# Autodesk Inventor assembly: Ensemble côté suspension
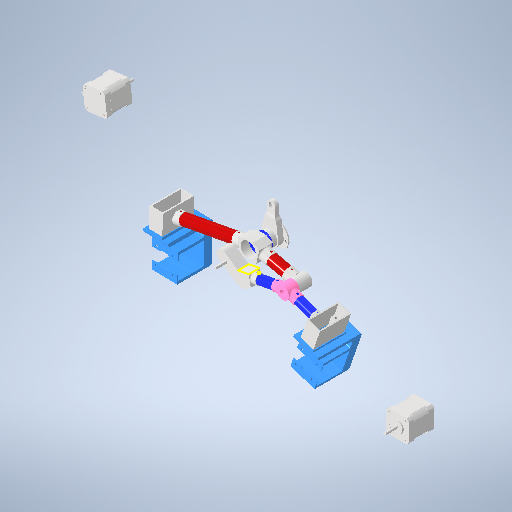
[picture p0: Inventor's stored thumbnail of the model, 512x512]
Saved by Autodesk Inventor 2026.2 (Build 302298010, 298A)
## iProperties
Created: 2026-03-16
Part Number: Ensemble côté suspension
Document SubType Name: Assembly
Designer: genon
Author: genon
## Documents named in this file (16)
- C:\Users\genon\Documents\Henallux Passerelle\Projet de conception\Cassini T-X\Inventor\Suspension\Ensemble côté suspension.iam
- C:\Users\genon\Documents\Henallux Passerelle\Projet de conception\Cassini T-X\Inventor\Suspension\bièlle côté.ipt
- C:\Users\genon\Documents\Henallux Passerelle\Projet de conception\Cassini T-X\Inventor\Suspension\bielle côté 2.ipt
- C:\Users\genon\Documents\Henallux Passerelle\Projet de conception\Cassini T-X\Inventor\Suspension\bielle côté 3.ipt
- C:\Users\genon\Documents\Henallux Passerelle\Projet de conception\Cassini T-X\Inventor\Suspension\bielle côté 0.ipt
- C:\Users\genon\Documents\Henallux Passerelle\Projet de conception\Cassini T-X\Inventor\Suspension\Rolling v2.ipt
- C:\Users\genon\Documents\Henallux Passerelle\Projet de conception\Cassini T-X\Inventor\Suspension\tubelong_rocker.ipt
- C:\Users\genon\Documents\Henallux Passerelle\Projet de conception\Cassini T-X\Inventor\Suspension\tube vers bogie.ipt
- C:\Users\genon\Documents\Henallux Passerelle\Projet de conception\Cassini T-X\Inventor\Suspension\bielle rocker.ipt
- C:\Users\genon\Documents\Henallux Passerelle\Projet de conception\Cassini T-X\Inventor\Suspension\bielle rocker2.ipt
- C:\Users\genon\Documents\Henallux Passerelle\Projet de conception\Cassini T-X\Inventor\Suspension\bielle roue milieu.ipt
- C:\Users\genon\Documents\Henallux Passerelle\Projet de conception\Cassini T-X\Inventor\Suspension\Attache moteur.ipt
- C:\Users\genon\Documents\Henallux Passerelle\Projet de conception\Cassini T-X\Inventor\Suspension\tube des bogies.ipt
- C:\Users\genon\Documents\Henallux Passerelle\Projet de conception\Cassini T-X\Inventor\Composants\NEMA17_17HS19-2004S1_Stepperonline.ipt
- C:\Users\genon\Documents\Henallux Passerelle\Projet de conception\Cassini T-X\Inventor\Suspension\Attache servomoteur.ipt
- C:\Users\genon\Documents\Henallux Passerelle\Projet de conception\Cassini T-X\Inventor\Suspension\Attache servomoteur_bogie.ipt
## Components (21 placed, 15 different names)
1. bièlle côté:1 — Placage:10, Placage:11, Placage:12, Placage:13, Placage:14, Placage:17, Placage:18, Placage:19
2. bielle côté 2:1 — Placage:8, Placage:9, Placage:15, Placage:16, Placage:17, Placage:18
3. bielle côté 3:1 — Placage:15, Placage:16, Cylindrique:1, Cylindrique:7, Placage:32, Placage:41
4. bielle côté 0:1 — Placage:12
5. Rolling v2:2 — Placage:8, Placage:9, Placage:19
6. Rolling v2:3 — Placage:10, Placage:11
7. bielle côté 0:2 — Placage:13, Placage:14
8. tubelong_rocker:1 — Cylindrique:1, Placage:41, Placage:42, Placage:43
9. tube vers bogie:1 — Cylindrique:7, Placage:32, Cylindrique:8, Placage:33
10. bielle rocker2:1 — Placage:31, Cylindrique:9, Placage:34, Cylindrique:10, Placage:35, Cylindrique:13
11. bielle roue milieu:1 — Cylindrique:11, Placage:36
12. bielle rocker:1 — Placage:29, Placage:31, Cylindrique:8, Placage:33, Cylindrique:12, Cylindrique:13
13. Rolling v2:4 — Placage:29, Cylindrique:12
14. tube des bogies:1 — Cylindrique:9, Placage:34, Cylindrique:11, Placage:36
15. tube des bogies:2 — Cylindrique:10, Placage:35, Placage:44, Placage:45
16. NEMA17_17HS19-2004S1_Stepperonline:1
17. NEMA17_17HS19-2004S1_Stepperonline:2
18. Attache servomoteur:1 — Placage:42, Placage:43, Placage:46, Placage:47, Placage:48
19. Attache servomoteur_bogie:1 — Placage:44, Placage:45, Placage:49, Placage:50, Placage:51
20. Attache moteur:1 — Placage:46, Placage:47, Placage:48
21. Attache moteur:2 — Placage:49, Placage:50, Placage:51
## Relationships (38: Mate 30, CylindricalJoint 8)
- Placage:8 [Mate]: bielle côté 2:1 ↔ Rolling v2:2
- Placage:9 [Mate]: bielle côté 2:1 ↔ Rolling v2:2
- Placage:10 [Mate]: bièlle côté:1 ↔ Rolling v2:3
- Placage:11 [Mate]: bièlle côté:1 ↔ Rolling v2:3
- Placage:12 [Mate]: bièlle côté:1 ↔ bielle côté 0:1
- Placage:13 [Mate]: bièlle côté:1 ↔ bielle côté 0:2
- Placage:14 [Mate]: bièlle côté:1 ↔ bielle côté 0:2
- Placage:15 [Mate]: bielle côté 2:1 ↔ bielle côté 3:1
- Placage:16 [Mate]: bielle côté 2:1 ↔ bielle côté 3:1
- Placage:17 [Mate]: bièlle côté:1 ↔ bielle côté 2:1
- Placage:18 [Mate]: bièlle côté:1 ↔ bielle côté 2:1
- Placage:19 [Mate]: bièlle côté:1 ↔ Rolling v2:2
- Cylindrique:1: bielle côté 3:1 ↔ tubelong_rocker:1
- Placage:29 [Mate]: bielle rocker:1 ↔ Rolling v2:4
- Placage:31 [Mate]: bielle rocker2:1 ↔ bielle rocker:1
- Cylindrique:7: bielle côté 3:1 ↔ tube vers bogie:1
- Placage:32 [Mate]: bielle côté 3:1 ↔ tube vers bogie:1
- Cylindrique:8: tube vers bogie:1 ↔ bielle rocker:1
- Placage:33 [Mate]: tube vers bogie:1 ↔ bielle rocker:1
- Cylindrique:9: bielle rocker2:1 ↔ tube des bogies:1
- Placage:34 [Mate]: bielle rocker2:1 ↔ tube des bogies:1
- Cylindrique:10: bielle rocker2:1 ↔ tube des bogies:2
- Placage:35 [Mate]: bielle rocker2:1 ↔ tube des bogies:2
- Cylindrique:11: bielle roue milieu:1 ↔ tube des bogies:1
- Placage:36 [Mate]: bielle roue milieu:1 ↔ tube des bogies:1
- Placage:41 [Mate]: bielle côté 3:1 ↔ tubelong_rocker:1
- Placage:42 [Mate]: tubelong_rocker:1 ↔ Attache servomoteur:1
- Placage:43 [Mate]: tubelong_rocker:1 ↔ Attache servomoteur:1
- Placage:44 [Mate]: tube des bogies:2 ↔ Attache servomoteur_bogie:1
- Placage:45 [Mate]: tube des bogies:2 ↔ Attache servomoteur_bogie:1
- Placage:46 [Mate]: Attache servomoteur:1 ↔ Attache moteur:1
- Placage:47 [Mate]: Attache servomoteur:1 ↔ Attache moteur:1
- Placage:48 [Mate]: Attache servomoteur:1 ↔ Attache moteur:1
- Placage:49 [Mate]: Attache servomoteur_bogie:1 ↔ Attache moteur:2
- Placage:50 [Mate]: Attache servomoteur_bogie:1 ↔ Attache moteur:2
- Placage:51 [Mate]: Attache servomoteur_bogie:1 ↔ Attache moteur:2
- Cylindrique:12: bielle rocker:1 ↔ Rolling v2:4
- Cylindrique:13: bielle rocker2:1 ↔ bielle rocker:1
